# Autodesk Inventor assembly: HEADERS HEMBR
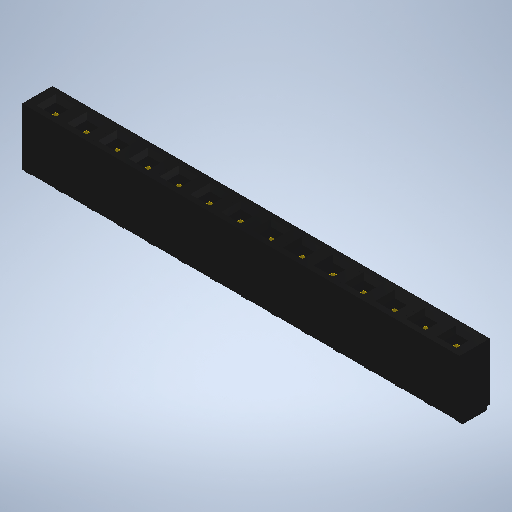
[picture p0: Inventor's stored thumbnail of the model, 512x512]
Saved by Autodesk Inventor 2025.2 (Build 292293000, 293)
## iProperties
Created: 2025-10-27
Part Number: HEADERS HEMBR
Material: Generic
Document SubType Name: Assembly
Designer: Ricardo
Author: Ricardo
## Documents named in this file (2)
- C:\Users\Ricardo\Documents\Inventor\TFC\Componentes\female-header-pins-2.snapshot.2\HEADERS HEMBR.iam
- C:\Users\Ricardo\Documents\Inventor\TFC\Componentes\female-header-pins-2.snapshot.2\2PINparEnsamble.ipt
## Components (7 placed, 1 different names)
1. 2PINparEnsamble:1 — Flush:1, Mate:1, Flush:2
2. 2PINparEnsamble:2 — Flush:1, Mate:1, Flush:2, Flush:3, Flush:4, Mate:2
3. 2PINparEnsamble:3 — Flush:3, Flush:4, Mate:2, Flush:5, Flush:6, Mate:3
4. 2PINparEnsamble:4 — Flush:5, Flush:6, Mate:3, Flush:7, Flush:8, Mate:4
5. 2PINparEnsamble:5 — Flush:7, Flush:8, Mate:4, Flush:9, Flush:10, Mate:5
6. 2PINparEnsamble:6 — Flush:9, Flush:10, Mate:5, Mate:6, Flush:11, Flush:12
7. 2PINparEnsamble:7 — Mate:6, Flush:11, Flush:12
## Relationships (18: Flush 12, Mate 6)
- Flush:1: 2PINparEnsamble:1 ↔ 2PINparEnsamble:2
- Mate:1 (-0.5 mm): 2PINparEnsamble:1 ↔ 2PINparEnsamble:2
- Flush:2: 2PINparEnsamble:1 ↔ 2PINparEnsamble:2
- Flush:3: 2PINparEnsamble:2 ↔ 2PINparEnsamble:3
- Flush:4: 2PINparEnsamble:2 ↔ 2PINparEnsamble:3
- Mate:2 (-0.5 mm): 2PINparEnsamble:2 ↔ 2PINparEnsamble:3
- Flush:5: 2PINparEnsamble:3 ↔ 2PINparEnsamble:4
- Flush:6: 2PINparEnsamble:3 ↔ 2PINparEnsamble:4
- Mate:3 (-0.5 mm): 2PINparEnsamble:3 ↔ 2PINparEnsamble:4
- Flush:7: 2PINparEnsamble:4 ↔ 2PINparEnsamble:5
- Flush:8: 2PINparEnsamble:4 ↔ 2PINparEnsamble:5
- Mate:4 (-0.5 mm): 2PINparEnsamble:4 ↔ 2PINparEnsamble:5
- Flush:9: 2PINparEnsamble:5 ↔ 2PINparEnsamble:6
- Flush:10: 2PINparEnsamble:5 ↔ 2PINparEnsamble:6
- Mate:5 (-0.5 mm): 2PINparEnsamble:5 ↔ 2PINparEnsamble:6
- Mate:6 (-0.5 mm): 2PINparEnsamble:6 ↔ 2PINparEnsamble:7
- Flush:11: 2PINparEnsamble:6 ↔ 2PINparEnsamble:7
- Flush:12: 2PINparEnsamble:6 ↔ 2PINparEnsamble:7
